# Autodesk Inventor assembly: Peristaltic pump adapter
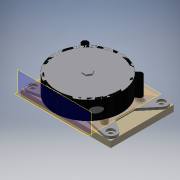
[picture p0: Inventor's stored thumbnail of the model, 180x180]
Saved by Autodesk Inventor 2017 (Build 210142000, 142)
## iProperties
Created: 2016-11-08
Part Number: Peristaltic pump adapter
Document SubType Name: Assembly
Designer: Camilo
Author: Camilo
## Documents named in this file (7)
- Z:\Github\AgingTests\3D parts\Peristaltic pump adapter\Peristaltic pump adapter.iam
- Z:\Github\AgingTests\3D parts\Peristaltic pump adapter\pumpHead.ipt
- Z:\Github\AgingTests\3D parts\Peristaltic pump adapter\adpaterPlate.ipt
- Z:\Github\AgingTests\3D parts\Peristaltic pump adapter\pumpSchematic.ipt
- Z:\Github\AgingTests\3D parts\Peristaltic pump adapter\dowel_M2.ipt
- Z:\Github\AgingTests\3D parts\Peristaltic pump adapter\peristalticPumpExtension.ipt
- Z:\Github\AgingTests\3D parts\Peristaltic pump adapter\rotor.ipt
## Components (7 placed, 6 different names)
1. pumpHead:1 — Flush:1
2. adpaterPlate:1 — Flush:1, Flush:2, Mate:1, Mate:2, Mate:3, Mate:4, Flush:4
3. pumpSchematic:1 — Flush:2, Flush:3
4. dowel_M2:1 — Mate:3, Mate:4
5. dowel_M2:2 — Mate:1, Mate:2
6. peristalticPumpExtension:1 — Flush:3
7. rotor:1 — Flush:4
## Relationships (8: Flush 4, Mate 4)
- Flush:1: pumpHead:1 ↔ adpaterPlate:1
- Flush:2: adpaterPlate:1 ↔ pumpSchematic:1
- Mate:1: adpaterPlate:1 ↔ dowel_M2:2
- Mate:2: adpaterPlate:1 ↔ dowel_M2:2
- Mate:3: adpaterPlate:1 ↔ dowel_M2:1
- Mate:4: adpaterPlate:1 ↔ dowel_M2:1
- Flush:3: pumpSchematic:1 ↔ peristalticPumpExtension:1
- Flush:4: adpaterPlate:1 ↔ rotor:1
